# Autodesk Inventor assembly: MotorArm_3D
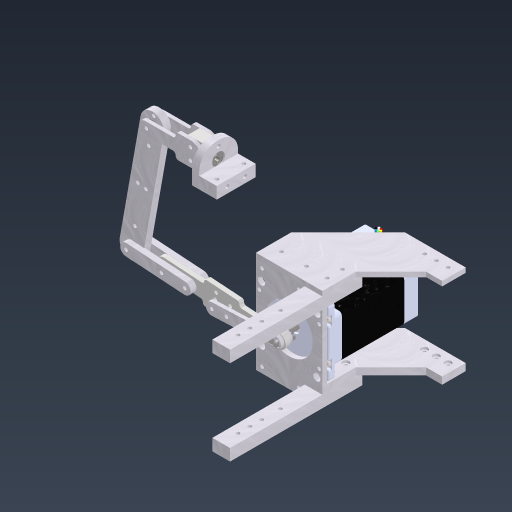
[picture p0: Inventor's stored thumbnail of the model, 512x512]
Saved by Autodesk Inventor 2023 (Build 270158000, 158)
## iProperties
Created: 2024-02-10
Part Number: MotorArm_3D
Document SubType Name: Assembly
Designer: victo
Author: victo
## Documents named in this file (18)
- C:\Users\victo\Documents\ball-balancing-digital-twin\Mechanics\CAD\MotorArm_3D.iam
- C:\Users\victo\Documents\ball-balancing-digital-twin\Mechanics\CAD\Step Motor Nema AK23 - 15kg.ipt
- C:\Users\victo\Documents\ball-balancing-digital-twin\Mechanics\CAD\motorAxis.ipt
- C:\Users\victo\Documents\ball-balancing-digital-twin\Mechanics\CAD\Arm1_3D.ipt
- C:\Users\victo\Documents\ball-balancing-digital-twin\Mechanics\CAD\Arm2_3D.ipt
- C:\Users\victo\Documents\ball-balancing-digital-twin\Mechanics\CAD\Arm3_3D.ipt
- C:\Users\victo\Documents\ball-balancing-digital-twin\Mechanics\CAD\bearing 1.ipt
- C:\Users\victo\Documents\ball-balancing-digital-twin\Mechanics\CAD\Arm4_3D.ipt
- C:\Users\victo\Documents\ball-balancing-digital-twin\Mechanics\CAD\Arm5_3D.ipt
- C:\Users\victo\Documents\ball-balancing-digital-twin\Mechanics\CAD\profile1_3D.ipt
- C:\Users\victo\Documents\ball-balancing-digital-twin\Mechanics\CAD\Arm6_3D.ipt
- C:\Users\victo\Documents\ball-balancing-digital-twin\Mechanics\CAD\profile2_3D.ipt
- C:\Users\victo\Documents\ball-balancing-digital-twin\Mechanics\CAD\MotorHolder_3D.ipt
- C:\Users\victo\Documents\ball-balancing-digital-twin\Mechanics\CAD\profile4_3D.ipt
- C:\Users\victo\Documents\ball-balancing-digital-twin\Mechanics\CAD\Plate_standard_3D.ipt
- C:\Users\victo\Documents\ball-balancing-digital-twin\Mechanics\CAD\Plate_Acrylic.ipt
- C:\Users\victo\Documents\ball-balancing-digital-twin\Mechanics\CAD\Plate_standard_low_3D.ipt
- C:\Users\victo\OneDrive\Documentos\Inventor\Content Center Files\R2023\en-US\ISO 4762(1)\DIN EN ISO 4762 - M3 x 12.ipt
## Components (25 placed, 17 different names)
1. Step Motor Nema AK23 - 15kg:1 — Rotational:1, Mate:36, Mate:37, Angle:5
2. motorAxis:1 — Rotational:1, Mate:1, Angle:1, Mate:2, Angle:2, Mate:4, Angle:3, Flush:1, Mate:35
3. Arm1_3D:1 — Mate:1, Angle:1, Mate:3, Mate:5, Mate:6, Mate:7, Mate:8, Mate:9, Mate:10, Mate:11, Mate:12, Mate:52
4. Arm2_3D:1 — Mate:2, Angle:2, Mate:3, Mate:6, Flush:1
5. Arm2_3D:2 — Mate:4, Angle:3, Mate:5, Mate:53
6. Arm3_3D:1 — Mate:10, Mate:11, Mate:12, Rotational:2
7. Arm3_3D:2 — Mate:7, Mate:8, Mate:9
8. bearing 1:1 — Rotational:2, Mate:13, Mate:14, Mate:15, Mate:16
9. Arm4_3D:1 — Mate:15, Mate:16, Mate:17, Rotational:3, Mate:19, Mate:20
10. Arm4_3D:2 — Mate:13, Mate:14, Mate:17, Mate:21
11. bearing 1:2 — Rotational:3, Mate:18
12. Arm5_3D:1 — Mate:19, Mate:20, Mate:22, Mate:23, Mate:24, Mate:25
13. Arm5_3D:2 — Mate:18, Mate:21, Mate:22
14. profile1_3D:1 — Mate:23, Mate:24, Mate:25, Mate:26, Mate:31
15. Arm6_3D:1 — Mate:26, Mate:27, Mate:28, Mate:30, Flush:2, Mate:31
16. Arm6_3D:2 — Mate:29, Mate:30, Flush:2, Mate:32, Mate:33, Mate:34
17. bearing 1:3 — Mate:27, Mate:28, Mate:29
18. profile2_3D:1 — Mate:32, Mate:33, Mate:34, Angle:5, Mate:43, Mate:44, Mate:45
19. MotorHolder_3D:1 — Mate:35, Mate:36, Mate:37, Mate:38, Angle:4, Mate:39, Mate:46, Mate:47, Mate:48
20. profile4_3D:1 — Mate:38, Angle:4, Mate:39, Mate:40, Mate:41, Mate:42
21. Plate_standard_3D:1 — Mate:40, Mate:41, Mate:42
22. Plate_Acrylic:1 — Mate:43, Mate:44, Mate:45
23. profile4_3D:2 — Mate:46, Mate:47, Mate:48, Mate:49, Mate:50, Mate:51
24. Plate_standard_low_3D:1 — Mate:49, Mate:50, Mate:51
25. DIN EN ISO 4762 M3 x 12:1 — Mate:52, Mate:53
## Relationships (63: Mate 53, Angle 5, RevoluteJoint 3, Flush 2)
- Rotational:1 [RevoluteJoint]: Step Motor Nema AK23 - 15kg:1 ↔ motorAxis:1
- Mate:1: motorAxis:1 ↔ Arm1_3D:1
- Angle:1 (180 deg): motorAxis:1 ↔ Arm1_3D:1
- Mate:2: motorAxis:1 ↔ Arm2_3D:1
- Angle:2 (180 deg): motorAxis:1 ↔ Arm2_3D:1
- Mate:3: Arm1_3D:1 ↔ Arm2_3D:1
- Mate:4: motorAxis:1 ↔ Arm2_3D:2
- Angle:3 (180 deg): motorAxis:1 ↔ Arm2_3D:2
- Mate:5: Arm1_3D:1 ↔ Arm2_3D:2
- Mate:6: Arm1_3D:1 ↔ Arm2_3D:1
- Mate:7: Arm1_3D:1 ↔ Arm3_3D:2
- Mate:8: Arm1_3D:1 ↔ Arm3_3D:2
- Mate:9 (1 mm): Arm1_3D:1 ↔ Arm3_3D:2
- Mate:10: Arm1_3D:1 ↔ Arm3_3D:1
- Mate:11: Arm1_3D:1 ↔ Arm3_3D:1
- Mate:12 (1 mm): Arm1_3D:1 ↔ Arm3_3D:1
- Flush:1: motorAxis:1 ↔ Arm2_3D:1
- Rotational:2 [RevoluteJoint] (-3.5 mm): Arm3_3D:1 ↔ bearing 1:1
- Mate:13: bearing 1:1 ↔ Arm4_3D:2
- Mate:14: bearing 1:1 ↔ Arm4_3D:2
- Mate:15: bearing 1:1 ↔ Arm4_3D:1
- Mate:16: bearing 1:1 ↔ Arm4_3D:1
- Mate:17: Arm4_3D:1 ↔ Arm4_3D:2
- Rotational:3 [RevoluteJoint]: Arm4_3D:1 ↔ bearing 1:2
- Mate:18: bearing 1:2 ↔ Arm5_3D:2
- Mate:19: Arm4_3D:1 ↔ Arm5_3D:1
- Mate:20 (2 mm): Arm4_3D:1 ↔ Arm5_3D:1
- Mate:21 (2 mm): Arm4_3D:2 ↔ Arm5_3D:2
- Mate:22: Arm5_3D:1 ↔ Arm5_3D:2
- Mate:23: Arm5_3D:1 ↔ profile1_3D:1
- Mate:24: Arm5_3D:1 ↔ profile1_3D:1
- Mate:25: Arm5_3D:1 ↔ profile1_3D:1
- Mate:26: profile1_3D:1 ↔ Arm6_3D:1
- Mate:27: Arm6_3D:1 ↔ bearing 1:3
- Mate:28: Arm6_3D:1 ↔ bearing 1:3
- Mate:29: Arm6_3D:2 ↔ bearing 1:3
- Mate:30: Arm6_3D:1 ↔ Arm6_3D:2
- Flush:2: Arm6_3D:1 ↔ Arm6_3D:2
- Mate:31: profile1_3D:1 ↔ Arm6_3D:1
- Mate:32: Arm6_3D:2 ↔ profile2_3D:1
- Mate:33: Arm6_3D:2 ↔ profile2_3D:1
- Mate:34: Arm6_3D:2 ↔ profile2_3D:1
- Mate:35: motorAxis:1 ↔ MotorHolder_3D:1
- Mate:36: Step Motor Nema AK23 - 15kg:1 ↔ MotorHolder_3D:1
- Mate:37: Step Motor Nema AK23 - 15kg:1 ↔ MotorHolder_3D:1
- Mate:38: MotorHolder_3D:1 ↔ profile4_3D:1
- Angle:4 (0 deg): MotorHolder_3D:1 ↔ profile4_3D:1
- Mate:39: MotorHolder_3D:1 ↔ profile4_3D:1
- Mate:40: profile4_3D:1 ↔ Plate_standard_3D:1
- Mate:41: profile4_3D:1 ↔ Plate_standard_3D:1
- Mate:42: profile4_3D:1 ↔ Plate_standard_3D:1
- Angle:5 (0 deg): Step Motor Nema AK23 - 15kg:1 ↔ profile2_3D:1
- Mate:43: profile2_3D:1 ↔ Plate_Acrylic:1
- Mate:44: profile2_3D:1 ↔ Plate_Acrylic:1
- Mate:45: profile2_3D:1 ↔ Plate_Acrylic:1
- Mate:46: MotorHolder_3D:1 ↔ profile4_3D:2
- Mate:47: MotorHolder_3D:1 ↔ profile4_3D:2
- Mate:48: MotorHolder_3D:1 ↔ profile4_3D:2
- Mate:49: profile4_3D:2 ↔ Plate_standard_low_3D:1
- Mate:50: profile4_3D:2 ↔ Plate_standard_low_3D:1
- Mate:51: profile4_3D:2 ↔ Plate_standard_low_3D:1
- Mate:52: Arm1_3D:1 ↔ DIN EN ISO 4762 M3 x 12:1
- Mate:53: Arm2_3D:2 ↔ DIN EN ISO 4762 M3 x 12:1
